# Autodesk Inventor assembly: sonsonmontajvidasız
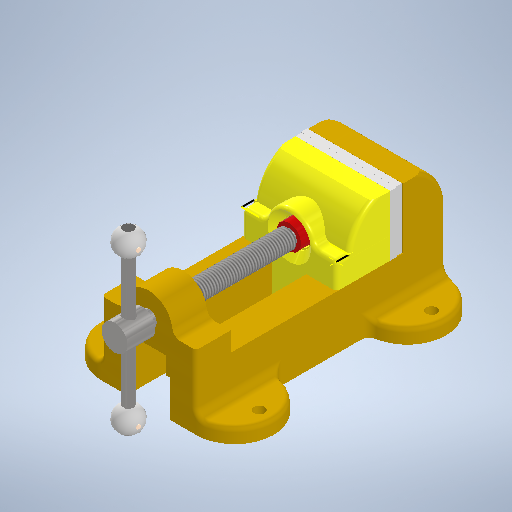
[picture p0: Inventor's stored thumbnail of the model, 512x512]
Saved by Autodesk Inventor 2025.4 (Build 294407000, 407)
## iProperties
Created: 2026-06-22
Part Number: sonsonmontajvidasız
Document SubType Name: Assembly
Designer: win10
Author: win10
## Documents named in this file (6)
- C:\Users\win10\Desktop\cad-final-projesi\sonsonmontajvidasız.iam
- C:\Users\win10\Desktop\cad-final-projesi\alt_plaka.ipt
- C:\Users\win10\Desktop\cad-final-projesi\haraketli_palaka.ipt
- C:\Users\win10\Desktop\cad-final-projesi\plaka.ipt
- C:\Users\win10\Documents\Inventor\Content Center Files\R2025\en-US\AS 1427(03)\AS 1427 - M6 x 16(1).ipt
- C:\Users\win10\Desktop\cad-final-projesi\VİDA_MİLİ2.iam
## Components (9 placed, 5 different names)
1. alt_plaka:1 — Mate:1, Mate:2, Insert:1, Insert:2, Mate:3
2. haraketli_palaka:1 — Mate:1, Mate:2, Insert:3, Insert:4, Mate:4
3. plaka:1 — Insert:1, Insert:2, Insert:7, Insert:8
4. plaka:2 — Insert:3, Insert:4, Insert:5, Insert:6
5. AS 1427 - Metric M6 x 16:1 — Insert:8
6. AS 1427 - Metric M6 x 16:2 — Insert:7
7. AS 1427 - Metric M6 x 16:3 — Insert:6
8. AS 1427 - Metric M6 x 16:4 — Insert:5
9. VİDA_MİLİ2:1 [sub-assembly] — Mate:3, Mate:4
## Relationships (12: Insert 8, Mate 4)
- Mate:1: alt_plaka:1 ↔ haraketli_palaka:1
- Mate:2: alt_plaka:1 ↔ haraketli_palaka:1
- Insert:1: alt_plaka:1 ↔ plaka:1
- Insert:2: alt_plaka:1 ↔ plaka:1
- Insert:3: haraketli_palaka:1 ↔ plaka:2
- Insert:4: haraketli_palaka:1 ↔ plaka:2
- Insert:5: plaka:2 ↔ AS 1427 - Metric M6 x 16:4
- Insert:6: plaka:2 ↔ AS 1427 - Metric M6 x 16:3
- Insert:7: plaka:1 ↔ AS 1427 - Metric M6 x 16:2
- Insert:8: plaka:1 ↔ AS 1427 - Metric M6 x 16:1
- Mate:3: alt_plaka:1 ↔ VİDA_MİLİ2:1
- Mate:4: haraketli_palaka:1 ↔ VİDA_MİLİ2:1
